# Autodesk Inventor assembly: Ensamblaje1
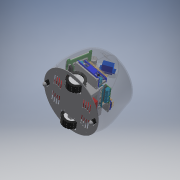
[picture p0: Inventor's stored thumbnail of the model, 180x180]
Saved by Autodesk Inventor 2018 (Build 220112000, 112)
## iProperties
Created: 2018-02-22
Part Number: Ensamblaje1
Material: Genérico
Document SubType Name: Assembly
Designer: ivanb
Author: ivanb
## Documents named in this file (22)
- C:\Users\ivanb\learnbot-git-annex\learnbot_desings\Learnbot2.1\IPT\Ensamblaje1.iam
- C:\Users\ivanb\learnbot-git-annex\learnbot_desings\Learnbot2.1\IPT\Base.ipt
- C:\Users\ivanb\learnbot-git-annex\learnbot_desings\Learnbot2.1\IPT\BackCase.ipt
- C:\Users\ivanb\learnbot-git-annex\learnbot_desings\Learnbot2.1\IPT\FrontCase.ipt
- C:\Users\ivanb\learnbot-git-annex\learnbot_desings\Learnbot2.0\filesToPrintLearnbot\IPT\carcasa_camara2.0.ipt
- C:\Users\ivanb\learnbot-git-annex\servo motor.ipt
- C:\Users\ivanb\learnbot-git-annex\learnbot_desings\Learnbot2.1\IPT\Wheel.ipt
- C:\Users\ivanb\learnbot-git-annex\learnbot_desings\Learnbot2.1\IPT\bola.ipt
- C:\Users\ivanb\learnbot-git-annex\learnbot_desings\Learnbot2.1\IPT\rueda servo.ipt
- C:\Users\ivanb\learnbot-git-annex\learnbot_desings\Learnbot2.1\IPT\tapa carcasa camara.ipt
- C:\Users\ivanb\learnbot-git-annex\learnbot_desings\raspberrypi.ipt
- C:\Users\ivanb\learnbot-git-annex\learnbot_desings\Learnbot2.1\IPT\baseRaspberry.ipt
- C:\Users\ivanb\learnbot-git-annex\learnbot_desings\Learnbot2.1\IPT\Pitft 3.5.ipt
- C:\Users\ivanb\learnbot-git-annex\learnbot_desings\Learnbot2.1\IPT\expansion.ipt
- C:\Users\ivanb\learnbot-git-annex\learnbot_desings\Learnbot2.1\IPT\Espaciador.ipt
- C:\Users\ivanb\learnbot-git-annex\learnbot_desings\Learnbot2.1\IPT\pololu 8835.ipt
- C:\Users\ivanb\learnbot-git-annex\learnbot_desings\Learnbot2.1\IPT\regulador de voltaje.ipt
- C:\Users\ivanb\learnbot-git-annex\learnbot_desings\Learnbot2.1\IPT\Espaciador19.5.ipt
- C:\Users\ivanb\learnbot-git-annex\learnbot_desings\Learnbot2.1\IPT\multiplicador de pines.ipt
- C:\Users\ivanb\learnbot-git-annex\learnbot_desings\Learnbot2.1\IPT\bateria.ipt
- C:\Users\ivanb\learnbot-git-annex\learnbot_desings\Learnbot2.1\IPT\Placa 16 pwm.ipt
- C:\Users\ivanb\learnbot-git-annex\learnbot_desings\Learnbot2.1\IPT\Soporte 16 pwm.ipt
## Components (27 placed, 21 different names)
1. Base:1 — Coincidencia:1, Insertar:1, Insertar:2, Coincidencia:2, Coincidencia:5, Coincidencia:6, Insertar:11, Insertar:12, Insertar:13, Insertar:14, Insertar:29, Insertar:30, Insertar:32, Insertar:33, Insertar:34, Insertar:35, Coincidencia:12
2. FrontCase:1 — Coincidencia:1, Insertar:1, Insertar:2, Insertar:6, Insertar:7, Insertar:8, Insertar:10, Insertar:19, Insertar:28, Insertar:29, Insertar:30, Coincidencia:14, Coincidencia:15, Coincidencia:16
3. BackCase:1 — Coincidencia:2, Insertar:32, Insertar:33
4. carcasa_camara2.0:1 — Nivelación:2, Insertar:8, Coincidencia:7, Insertar:9, Insertar:10, Insertar:19, Rígido:3, Insertar:20
5. servo motor:1 — Nivelación:2, Insertar:6, Insertar:7, De rotación:1, Insertar:28
6. Wheel:1 — Rígido:5
7. Wheel:2 — Rígido:4
8. bola:1 — Coincidencia:6, Insertar:11, Insertar:12
9. bola:2 — Coincidencia:5, Insertar:13, Insertar:14
10. rueda servo:1 — De rotación:1
11. tapa carcasa camara:1 — Coincidencia:7, Insertar:9, Rígido:3, Insertar:20
12. Pitft 3.5:1 — Coincidencia:14, Coincidencia:15, Coincidencia:16
13. baseRaspberry:1 — Insertar:34, Insertar:35, Rígido:4, Rígido:5, Insertar:36, Insertar:37, Insertar:50, Insertar:51, Coincidencia:13
14. raspberrypi:1 — Insertar:36, Insertar:37, Tangente:1, Tangente:2, Coincidencia:10, Insertar:38, Insertar:39, Insertar:40, Insertar:41
15. expansion:1 — Tangente:1, Tangente:2, Coincidencia:10, Coincidencia:11, Rígido:6, Insertar:52, Insertar:53
16. Espaciador:1 — Insertar:38
17. Espaciador:2 — Insertar:39
18. Espaciador:3 — Insertar:41
19. Espaciador:4 — Insertar:40
20. pololu 8835:1 — Coincidencia:11, Rígido:6
21. regulador de voltaje:1 — Insertar:46, Insertar:47, Insertar:50, Insertar:51
22. Espaciador19.5:3 — Insertar:46, Insertar:48
23. Espaciador19.5:4 — Insertar:47, Insertar:49
24. multiplicador de pines:1 — Insertar:48, Insertar:49
25. bateria:1 — Coincidencia:12, Coincidencia:13
26. Placa 16 pwm:1 — Insertar:54, Insertar:55
27. Soporte 16 pwm:1 — Insertar:52, Insertar:53, Insertar:54, Insertar:55
## Relationships (56: Insert 36, Mate 12, WeldJoint 4, Tangent 2, Flush 1, RevoluteJoint 1)
- Coincidencia:1 [Mate]: Base:1 ↔ FrontCase:1
- Insertar:1: Base:1 ↔ FrontCase:1
- Insertar:2: Base:1 ↔ FrontCase:1
- Coincidencia:2 [Mate]: Base:1 ↔ BackCase:1
- Nivelación:2 [Flush]: carcasa_camara2.0:1 ↔ servo motor:1
- Insertar:6: FrontCase:1 ↔ servo motor:1
- Insertar:7: FrontCase:1 ↔ servo motor:1
- Coincidencia:5 [Mate]: Base:1 ↔ bola:2
- Coincidencia:6 [Mate]: Base:1 ↔ bola:1
- Insertar:8: FrontCase:1 ↔ carcasa_camara2.0:1
- De rotación:1 [RevoluteJoint]: servo motor:1 ↔ rueda servo:1
- Coincidencia:7 [Mate]: carcasa_camara2.0:1 ↔ tapa carcasa camara:1
- Insertar:9: carcasa_camara2.0:1 ↔ tapa carcasa camara:1
- Insertar:10: FrontCase:1 ↔ carcasa_camara2.0:1
- Insertar:11: Base:1 ↔ bola:1
- Insertar:12: Base:1 ↔ bola:1
- Insertar:13: Base:1 ↔ bola:2
- Insertar:14: Base:1 ↔ bola:2
- Insertar:19: FrontCase:1 ↔ carcasa_camara2.0:1
- Rígido:3 [WeldJoint]: carcasa_camara2.0:1 ↔ tapa carcasa camara:1
- Insertar:20: carcasa_camara2.0:1 ↔ tapa carcasa camara:1
- Insertar:28: FrontCase:1 ↔ servo motor:1
- Insertar:29: Base:1 ↔ FrontCase:1
- Insertar:30: Base:1 ↔ FrontCase:1
- Insertar:32: Base:1 ↔ BackCase:1
- Insertar:33: Base:1 ↔ BackCase:1
- Insertar:34: Base:1 ↔ baseRaspberry:1
- Insertar:35: Base:1 ↔ baseRaspberry:1
- Rígido:4 [WeldJoint]: Wheel:2 ↔ baseRaspberry:1
- Rígido:5 [WeldJoint]: Wheel:1 ↔ baseRaspberry:1
- Insertar:36: baseRaspberry:1 ↔ raspberrypi:1
- Insertar:37: baseRaspberry:1 ↔ raspberrypi:1
- Tangente:1: raspberrypi:1 ↔ expansion:1
- Tangente:2: raspberrypi:1 ↔ expansion:1
- Coincidencia:10 [Mate]: raspberrypi:1 ↔ expansion:1
- Insertar:38: raspberrypi:1 ↔ Espaciador:1
- Insertar:39: raspberrypi:1 ↔ Espaciador:2
- Insertar:40: raspberrypi:1 ↔ Espaciador:4
- Insertar:41: raspberrypi:1 ↔ Espaciador:3
- Coincidencia:11 [Mate]: expansion:1 ↔ pololu 8835:1
- Rígido:6 [WeldJoint]: expansion:1 ↔ pololu 8835:1
- Insertar:46: regulador de voltaje:1 ↔ Espaciador19.5:3
- Insertar:47: regulador de voltaje:1 ↔ Espaciador19.5:4
- Insertar:48: Espaciador19.5:3 ↔ multiplicador de pines:1
- Insertar:49: Espaciador19.5:4 ↔ multiplicador de pines:1
- Insertar:50: baseRaspberry:1 ↔ regulador de voltaje:1
- Insertar:51: baseRaspberry:1 ↔ regulador de voltaje:1
- Coincidencia:12 [Mate]: Base:1 ↔ bateria:1
- Coincidencia:13 [Mate]: baseRaspberry:1 ↔ bateria:1
- Coincidencia:14 [Mate]: FrontCase:1 ↔ Pitft 3.5:1
- Coincidencia:15 [Mate]: FrontCase:1 ↔ Pitft 3.5:1
- Coincidencia:16 [Mate]: FrontCase:1 ↔ Pitft 3.5:1
- Insertar:52: expansion:1 ↔ Soporte 16 pwm:1
- Insertar:53: expansion:1 ↔ Soporte 16 pwm:1
- Insertar:54: Placa 16 pwm:1 ↔ Soporte 16 pwm:1
- Insertar:55: Placa 16 pwm:1 ↔ Soporte 16 pwm:1
